# Autodesk Inventor assembly: stacked
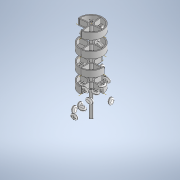
[picture p0: Inventor's stored thumbnail of the model, 180x180]
Saved by Autodesk Inventor 2022 (Build 260153000, 153)
## iProperties
Created: 2022-03-07
Part Number: stacked
Document SubType Name: Assembly
Designer: Alicia
Author: Alicia
## Documents named in this file (8)
- C:\Users\Public\Documents\Autodesk\Inventor 2022\Dispenser\Plan B Design\print files\stacked.iam
- C:\Users\Public\Documents\Autodesk\Inventor 2022\Dispenser\Plan B Design\base layer 1.ipt
- C:\Users\Public\Documents\Autodesk\Inventor 2022\Dispenser\Plan B Design\wheel of the walls.ipt
- C:\Users\Public\Documents\Autodesk\Inventor 2022\Dispenser\Plan B Design\base layer 2.ipt
- C:\Users\Public\Documents\Autodesk\Inventor 2022\Dispenser\Plan B Design\base layer 3.ipt
- C:\Users\Public\Documents\Autodesk\Inventor 2022\Dispenser\Plan B Design\base layer 4.ipt
- C:\Users\Public\Documents\Autodesk\Inventor 2022\Dispenser\Plan B Design\print files\shaft.ipt
- C:\Users\Public\Documents\Autodesk\Inventor 2022\Dispenser\Plan B Design\pill.ipt
## Components (31 placed, 7 different names)
1. base layer 1:1 — Mate:1, Mate:2, Rotational:1, Mate:24, Mate:25
2. wheel of the walls:1 — Mate:3, Rotational:1
3. base layer 2:1 — Mate:4, Mate:5, Mate:6, Rotational:2, Mate:22, Mate:23
4. wheel of the walls:2 — Mate:6, Rotational:2
5. base layer 3:1 — Mate:7, Mate:8, Rotational:3, Mate:20, Mate:21
6. wheel of the walls:3 — Mate:9, Rotational:3
7. base layer 4:1 — Mate:10, Mate:11, Rotational:4, Mate:18, Mate:19
8. wheel of the walls:4 — Mate:12, Rotational:4, Rigid:1
9. shaft:1 — Mate:13, Rigid:1
10. pill:1 — Mate:20
11. pill:2 — Mate:18
12. pill:3
13. pill:4
14. pill:5 — Mate:23
15. pill:6
16. pill:7
17. pill:8 — Mate:24
18. pill:9
19. pill:10
20. pill:11
21. pill:12
22. pill:14 — Mate:25
23. pill:15
24. pill:17 — Mate:21
25. pill:18
26. pill:19
27. pill:20
28. pill:21 — Mate:22
29. pill:22 — Mate:19
30. pill:23
31. pill:24
## Relationships (29: Mate 21, RevoluteJoint 4, Flush 3, WeldJoint 1)
- Mate:1: base layer 1:1
- Mate:2: base layer 1:1
- Mate:3: wheel of the walls:1
- Rotational:1 [RevoluteJoint]: base layer 1:1 ↔ wheel of the walls:1
- Flush:1 (30 mm)
- Mate:4: base layer 2:1
- Mate:5: base layer 2:1
- Mate:6: base layer 2:1 ↔ wheel of the walls:2
- Rotational:2 [RevoluteJoint]: base layer 2:1 ↔ wheel of the walls:2
- Flush:2 (60 mm)
- Mate:7: base layer 3:1
- Mate:8: base layer 3:1
- Mate:9: wheel of the walls:3
- Rotational:3 [RevoluteJoint]: base layer 3:1 ↔ wheel of the walls:3
- Flush:3 (90 mm)
- Mate:10: base layer 4:1
- Mate:11: base layer 4:1
- Mate:12: wheel of the walls:4
- Rotational:4 [RevoluteJoint]: base layer 4:1 ↔ wheel of the walls:4
- Mate:13: shaft:1
- Rigid:1 [WeldJoint]: wheel of the walls:4 ↔ shaft:1
- Mate:18: base layer 4:1 ↔ pill:2
- Mate:19: base layer 4:1 ↔ pill:22
- Mate:20: base layer 3:1 ↔ pill:1
- Mate:21: base layer 3:1 ↔ pill:17
- Mate:22: base layer 2:1 ↔ pill:21
- Mate:23: base layer 2:1 ↔ pill:5
- Mate:24: base layer 1:1 ↔ pill:8
- Mate:25: base layer 1:1 ↔ pill:14
